# Autodesk Inventor assembly: Laminated Board
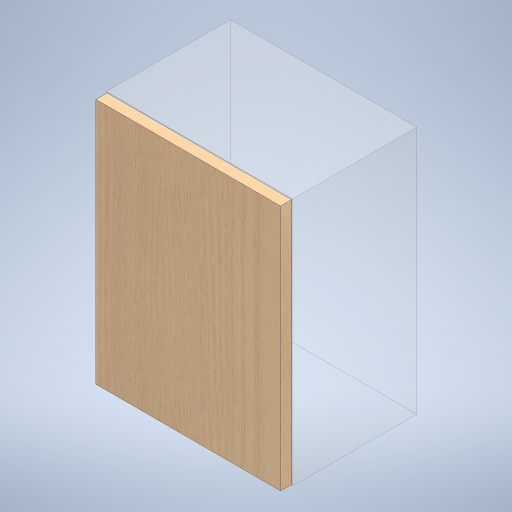
[picture p0: Inventor's stored thumbnail of the model, 512x512]
Saved by Autodesk Inventor 2024 (Build 280153000, 153)
## iProperties
RuleStatus: InUse
Created: 2014-05-07
Part Number: Laminated Board
Document SubType Name: Assembly
Designer: SauliusD
Description: Laminated Board Facade
Author: SauliusD
## Documents named in this file (3)
- C:\W4INV 2024 Design\iBOX LIBRARY\Facades\Laminated Board Facade\Laminated Board Facade.iam
- C:\W4INV 2024 Design\iBOX LIBRARY\Facades\Laminated Board Facade\Laminated Board Facade.ipt
- C:\W4INV 2024 Design\iBOX LIBRARY\Facades\Laminated Board Facade\Laminated Board Facade Skeleton.ipt
## Components (2 placed, 2 different names)
1. @Skeleton — Flush:4, Flush:5, Flush:6
2. Laminated Board Facade:1 — Flush:1, Flush:2, Flush:3
## Relationships (6: Flush 6)
- Flush:1: Laminated Board Facade:1
- Flush:2: Laminated Board Facade:1
- Flush:3: Laminated Board Facade:1
- Flush:4: @Skeleton
- Flush:5: @Skeleton
- Flush:6: @Skeleton
## Named parameters: Offset_From_Left = 1.5 mm, Offset_From_Right = 1.5 mm, Offset_From_Top = 1.5 mm, Offset_From_Bottom = 1.5 mm, Panel_Thickness = 18 mm
